# Autodesk Inventor assembly: subflap
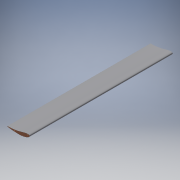
[picture p0: Inventor's stored thumbnail of the model, 180x180]
Saved by Autodesk Inventor 2018.2 (Build 222227000, 227)
## iProperties
Created: 2018-03-14
Part Number: subflap
Material: 一般
Document SubType Name: Assembly
Designer: ku_sk
Author: ku_sk
## Documents named in this file (4)
- D:\ku_sk\ドキュメント\Inventor\Aero\KS-15\Rr.wing\parts\subflap\subflap.iam
- D:\ku_sk\ドキュメント\Inventor\Aero\KS-15\Rr.wing\parts\subflap\parts\flap_s.ipt
- D:\ku_sk\ドキュメント\Inventor\Aero\KS-15\Rr.wing\parts\subflap\parts\uretan_s.ipt
- D:\ku_sk\ドキュメント\Inventor\Aero\KS-15\Rr.wing\parts\subflap\parts\GFRP_sub.ipt
## Components (10 placed, 3 different names)
1. flap_s:1 — メイト:2, メイト:11, メイト:12, メイト:14, メイト:18, メイト:19, メイト:20, メイト:21, メイト:22, メイト:23, メイト:27, フラッシュ:2
2. flap_s:2 — メイト:1, メイト:2, メイト:9, メイト:10, メイト:11, メイト:12, メイト:15
3. flap_s:3 — メイト:1, メイト:3, メイト:5, メイト:6, メイト:9, メイト:10, フラッシュ:1, 角度:1, メイト:13, メイト:16
4. flap_s:4 — メイト:3, メイト:4, メイト:5, メイト:6, メイト:7, メイト:8, メイト:17, メイト:24
5. flap_s:5 — メイト:4, メイト:7, メイト:8, メイト:25
6. uretan_s:1 — メイト:17, メイト:21, メイト:25
7. uretan_s:2 — メイト:16, メイト:20, メイト:24
8. uretan_s:3 — メイト:15, メイト:19, メイト:23, メイト:26
9. uretan_s:4 — メイト:14, メイト:18, メイト:22
10. GFRP_sub:1 — メイト:26, メイト:27, フラッシュ:2
## Relationships (30: Mate 27, Flush 2, Angle 1)
- メイト:1 [Mate] (41.5 mm): flap_s:2 ↔ flap_s:3
- メイト:2 [Mate] (41.5 mm): flap_s:1 ↔ flap_s:2
- メイト:3 [Mate] (41.5 mm): flap_s:3 ↔ flap_s:4
- メイト:4 [Mate] (41.5 mm): flap_s:4 ↔ flap_s:5
- メイト:5 [Mate]: flap_s:3 ↔ flap_s:4
- メイト:6 [Mate]: flap_s:3 ↔ flap_s:4
- メイト:7 [Mate]: flap_s:4 ↔ flap_s:5
- メイト:8 [Mate]: flap_s:4 ↔ flap_s:5
- メイト:9 [Mate]: flap_s:2 ↔ flap_s:3
- メイト:10 [Mate]: flap_s:2 ↔ flap_s:3
- メイト:11 [Mate]: flap_s:1 ↔ flap_s:2
- メイト:12 [Mate]: flap_s:1 ↔ flap_s:2
- フラッシュ:1 [Flush]: flap_s:3
- 角度:1 [Angle] (0 deg): flap_s:3
- メイト:13 [Mate]: flap_s:3
- メイト:14 [Mate]: flap_s:1 ↔ uretan_s:4
- メイト:15 [Mate]: flap_s:2 ↔ uretan_s:3
- メイト:16 [Mate]: flap_s:3 ↔ uretan_s:2
- メイト:17 [Mate]: flap_s:4 ↔ uretan_s:1
- メイト:18 [Mate]: flap_s:1 ↔ uretan_s:4
- メイト:19 [Mate]: flap_s:1 ↔ uretan_s:3
- メイト:20 [Mate]: flap_s:1 ↔ uretan_s:2
- メイト:21 [Mate]: flap_s:1 ↔ uretan_s:1
- メイト:22 [Mate]: flap_s:1 ↔ uretan_s:4
- メイト:23 [Mate]: flap_s:1 ↔ uretan_s:3
- メイト:24 [Mate]: flap_s:4 ↔ uretan_s:2
- メイト:25 [Mate]: flap_s:5 ↔ uretan_s:1
- メイト:26 [Mate]: uretan_s:3 ↔ GFRP_sub:1
- メイト:27 [Mate]: flap_s:1 ↔ GFRP_sub:1
- フラッシュ:2 [Flush]: flap_s:1 ↔ GFRP_sub:1
